# Autodesk Inventor assembly: 3030_connector_assembled
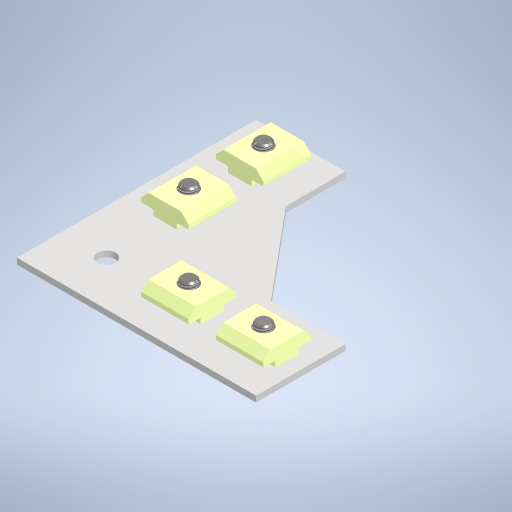
[picture p0: Inventor's stored thumbnail of the model, 512x512]
Saved by Autodesk Inventor 2024 (Build 280153000, 153)
## iProperties
Created: 2025-12-08
Part Number: 3030_connector_assembled
Document SubType Name: Assembly
Designer: schar
Author: schar
## Documents named in this file (4)
- C:\Users\schar\Desktop\projectBlueprint\AMSTS\hardware\3030_connector_assembled.iam
- C:\Users\schar\Desktop\projectBlueprint\AMSTS\hardware\Connect2x3030_m6.ipt
- C:\Users\schar\Desktop\projectBlueprint\AMSTS\hardware\3030_tnut_m6.ipt
- C:\Users\schar\Documents\Inventor\Content Center Files\R2024\en-US\AS 1420\AS 1420 - 1973 - M5 x 10.ipt
## Components (9 placed, 3 different names)
1. Connect2x3030_m6:1
2. 3030_tnut_m6:1
3. 3030_tnut_m6:2
4. 3030_tnut_m6:3
5. 3030_tnut_m6:4
6. AS 1420 - Metric M5 x 10:1
7. AS 1420 - Metric M5 x 10:2
8. AS 1420 - Metric M5 x 10:3
9. AS 1420 - Metric M5 x 10:4
## Relationships (8: RevoluteJoint 4, Insert 4)
- [RevoluteJoint] (-0.357 mm): Connect2x3030_m6:1 ↔ 3030_tnut_m6:3
- [RevoluteJoint] (-0.357 mm): Connect2x3030_m6:1 ↔ 3030_tnut_m6:4
- [RevoluteJoint] (-0.357 mm): Connect2x3030_m6:1 ↔ 3030_tnut_m6:2
- [RevoluteJoint] (-0.357 mm): Connect2x3030_m6:1 ↔ 3030_tnut_m6:1
- [Insert]: Connect2x3030_m6:1 ↔ AS 1420 - Metric M5 x 10:1
- [Insert]: Connect2x3030_m6:1 ↔ AS 1420 - Metric M5 x 10:2
- [Insert]: Connect2x3030_m6:1 ↔ AS 1420 - Metric M5 x 10:3
- [Insert]: Connect2x3030_m6:1 ↔ AS 1420 - Metric M5 x 10:4
## Named parameters: d198_d171 = 0 mm, d199_d172 = 0 mm, d200_d173 = 0 mm, d201_d174 = 0 mm, d202_d175 = 0 mm, d203_d176 = 0 mm, d204_d177 = 0 mm, d205_d178 = 0 mm, d206_d179 = 0 mm, d207_d183 = 0 mm, d208_d184 = 0 mm, d209_d185 = 0 mm, d210_d113 = 0 deg, d211_d114 = -0.357 mm, d212_d115 = 0 deg, d213_d116 = -0.357 mm, d214_d117 = 0 deg, d215_d110 = -0.357 mm, d216_d111 = 0 deg, d217_d112 = -0.357 mm
